# Autodesk Inventor assembly: DEWALT
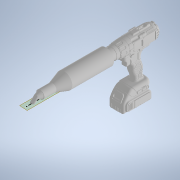
[picture p0: Inventor's stored thumbnail of the model, 180x180]
Saved by Autodesk Inventor 2022 (Build 260153000, 153)
## iProperties
Company: none
Created: 2011-08-21
Part Number: DEWALT
Description: CATIA V5 STEP Exchange
Document SubType Name: Assembly
Designer: Admin
Authority: none
Sending System: CATIA V5 STEP AP203
Preprocessor: CATIA Version 5 Release 20 GA (IN-10)
Title: F:\MUSTERILER\DeWALT\NEW\DEWALT_EDIT.stp
Author: none
## iProperties of the stored document MemberDocs/xAaaaabdaAaaaaaaaAaaaq5mfAg
Company: none
Created: 2011-08-21
Part Number: DEWALT
Description: CATIA V5 STEP Exchange
Document SubType Name: Assembly
Designer: Admin
Authority: none
Sending System: CATIA V5 STEP AP203
Preprocessor: CATIA Version 5 Release 20 GA (IN-10)
Title: F:\MUSTERILER\DeWALT\NEW\DEWALT_EDIT.stp
Author: none
## Documents named in this file (22)
- C:\Users\acer\Downloads\DEWALT-2 (1) (1)\DEWALT\DEWALT.iam
- C:\Users\acer\Downloads\DEWALT-2 (1) (1)\DEWALT\Part1.2.ipt
- C:\Users\acer\Downloads\DEWALT-2 (1) (1)\DEWALT\Part1.1.ipt
- C:\Users\acer\Downloads\DEWALT-2 (1) (1)\DEWALT\Part1.3.ipt
- C:\Users\acer\Downloads\DEWALT-2 (1) (1)\DEWALT\Part1.4.ipt
- C:\Users\acer\Downloads\DEWALT-2 (1) (1)\DEWALT\Part1.5.ipt
- C:\Users\acer\Downloads\DEWALT-2 (1) (1)\DEWALT\Part1.6.ipt
- C:\Users\acer\Downloads\DEWALT-2 (1) (1)\DEWALT\Part1.7.ipt
- C:\Users\acer\Downloads\DEWALT-2 (1) (1)\DEWALT\Part1.8.ipt
- C:\Users\acer\Downloads\DEWALT-2 (1) (1)\DEWALT\Part1.9.ipt
- C:\Users\acer\Downloads\DEWALT-2 (1) (1)\DEWALT\Part1.10.ipt
- C:\Users\acer\Downloads\DEWALT-2 (1) (1)\DEWALT\Part1.11.ipt
- C:\Users\acer\Downloads\DEWALT-2 (1) (1)\DEWALT\Part1.12.ipt
- C:\Users\acer\Downloads\DEWALT-2 (1) (1)\DEWALT\Part1.13.ipt
- C:\Users\acer\Downloads\DEWALT-2 (1) (1)\DEWALT\Part1.14.ipt
- C:\Users\acer\Downloads\DEWALT-2 (1) (1)\DEWALT\Part1.15.ipt
- C:\Users\acer\Downloads\DEWALT-2 (1) (1)\DEWALT\Part1.16.ipt
- C:\Users\acer\Downloads\DEWALT-2 (1) (1)\DEWALT\Product1.iam
- C:\Users\acer\Downloads\DEWALT-2 (1) (1)\DEWALT\Pièce35.ipt
- C:\Users\acer\Downloads\DEWALT-2 (1) (1)\DEWALT\impeller-pump-in-autodesk-inventor-inventor-3d-drawing-practice-tutorial-for-beginners-3d-cad-1.snapshot.1\Part2.ipt
- C:\Users\acer\Downloads\DEWALT-2 (1) (1)\DEWALT\Engine Air Filter.ipt
- C:\Users\acer\Downloads\DEWALT-2 (1) (1)\DEWALT\Pièce1.ipt
## Components (21 placed, 21 different names)
1. Part1.1
2. Part1.2
3. Part1.3
4. Part1.4
5. Part1.5
6. Part1.6
7. Part1.7 — Placage:1, Placage:6
8. Part1.8
9. Part1.9
10. Part1.10
11. Part1.11
12. Part1.12
13. Part1.13
14. Part1.14
15. Part1.15
16. Part1.16
17. Product1.1 [sub-assembly]
18. Pièce35:1 — Logement:1, Placage:1, Placage:2, Placage:4, Placage:5
19. Part2:1 — Logement:1, Placage:3, Placage:6
20. Engine Air Filter:1 — Placage:2, Placage:3
21. Pièce1:1 — Placage:4, Placage:5
## Relationships (7: Mate 6, Insert 1)
- Logement:1 [Insert]: Pièce35:1 ↔ Part2:1
- Placage:1 [Mate]: Part1.7 ↔ Pièce35:1
- Placage:2 [Mate]: Pièce35:1 ↔ Engine Air Filter:1
- Placage:3 [Mate] (10 mm): Part2:1 ↔ Engine Air Filter:1
- Placage:4 [Mate]: Pièce35:1 ↔ Pièce1:1
- Placage:5 [Mate]: Pièce35:1 ↔ Pièce1:1
- Placage:6 [Mate]: Part1.7 ↔ Part2:1
